# Autodesk Inventor assembly: CORL_007_PlanetaryGearbox
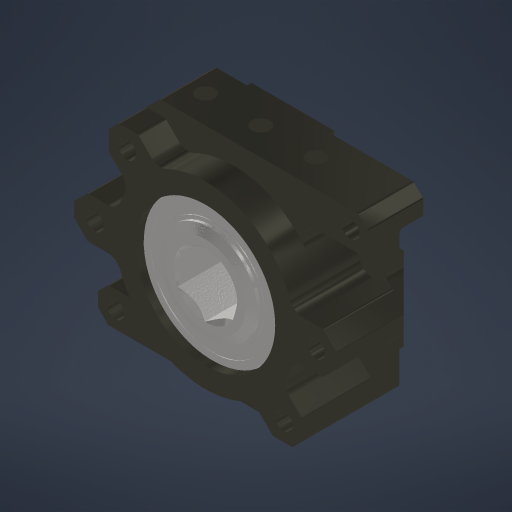
[picture p0: Inventor's stored thumbnail of the model, 512x512]
Saved by Autodesk Inventor 2024.2 (Build 282272000, 272)
## iProperties
Created: 2024-08-02
Part Number: CORL_007_PlanetaryGearbox
Document SubType Name: Assembly
Designer: Bryan
Author: Bryan
## Documents named in this file (6)
- C:\Users\bobsb\OneDrive\Documents\GitHub\1622-2024-Summer-CAD-A-Thon\Coral\CORL_007_PlanetaryGearbox.iam
- C:\Users\bobsb\OneDrive\Documents\GitHub\1622-2024-Summer-CAD-A-Thon\COTS Library\MAXPlanetary System\COTS_0.5inhexoutput_REV-21-2104.ipt
- C:\Users\bobsb\OneDrive\Documents\GitHub\1622-2024-Summer-CAD-A-Thon\COTS Library\MAXPlanetary System\COTS_3to1Stage_REV-21-2101.ipt
- C:\Users\bobsb\OneDrive\Documents\GitHub\1622-2024-Summer-CAD-A-Thon\COTS Library\MAXPlanetary System\COTS_InputStage_REV-21-2106.ipt
- C:\Users\bobsb\OneDrive\Documents\GitHub\1622-2024-Summer-CAD-A-Thon\COTS Library\MAXPlanetary System\COTS_NeoShaftAdapter_REV-21-2108.ipt
- C:\Users\bobsb\OneDrive\Documents\GitHub\1622-2024-Summer-CAD-A-Thon\COTS Library\Motors\COTS_REV-21-1650-V1.1_Neo1.1.ipt
## Components (5 placed, 5 different names)
1. COTS_0.5inhexoutput_REV-21-2104:1 — Mate:1, Mate:4, Flush:1
2. COTS_3to1Stage_REV-21-2101:1 — Mate:1, Mate:2, Mate:3, Mate:4, Flush:1, Flush:2, Mate:6
3. COTS_InputStage_REV-21-2106:1 — Mate:5, Flush:2, Mate:6, Mate:8, Mate:9
4. COTS_NeoShaftAdapter_REV-21-2108:1 — Mate:2, Mate:3, Mate:5, Mate:7
5. COTS_REV-21-1650-V1.1_Neo1.1:1 — Mate:7, Mate:8, Mate:9
## Relationships (11: Mate 9, Flush 2)
- Mate:1: COTS_0.5inhexoutput_REV-21-2104:1 ↔ COTS_3to1Stage_REV-21-2101:1
- Mate:2: COTS_3to1Stage_REV-21-2101:1 ↔ COTS_NeoShaftAdapter_REV-21-2108:1
- Mate:3: COTS_3to1Stage_REV-21-2101:1 ↔ COTS_NeoShaftAdapter_REV-21-2108:1
- Mate:4: COTS_0.5inhexoutput_REV-21-2104:1 ↔ COTS_3to1Stage_REV-21-2101:1
- Mate:5: COTS_InputStage_REV-21-2106:1 ↔ COTS_NeoShaftAdapter_REV-21-2108:1
- Flush:1: COTS_0.5inhexoutput_REV-21-2104:1 ↔ COTS_3to1Stage_REV-21-2101:1
- Flush:2: COTS_3to1Stage_REV-21-2101:1 ↔ COTS_InputStage_REV-21-2106:1
- Mate:6: COTS_3to1Stage_REV-21-2101:1 ↔ COTS_InputStage_REV-21-2106:1
- Mate:7: COTS_NeoShaftAdapter_REV-21-2108:1 ↔ COTS_REV-21-1650-V1.1_Neo1.1:1
- Mate:8: COTS_InputStage_REV-21-2106:1 ↔ COTS_REV-21-1650-V1.1_Neo1.1:1
- Mate:9: COTS_InputStage_REV-21-2106:1 ↔ COTS_REV-21-1650-V1.1_Neo1.1:1
